# Autodesk Inventor assembly: Planktoscope_Mini_v0
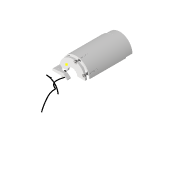
[picture p0: Inventor's stored thumbnail of the model, 180x180]
Saved by Autodesk Inventor 2022 (Build 260153000, 153)
## iProperties
Created: 2022-04-02
Part Number: Planktoscope_Mini_v0
Document SubType Name: Assembly
Designer: Prakash Lab
Author: Prakash Lab
## Documents named in this file (13)
- C:\Users\diederichbenedict\Dropbox\Dokumente\Promotion\PROJECTS\Matchboxscope\INVENTOR\Planktoscope_Mini\Planktoscope_Mini_v0.iam
- C:\Users\diederichbenedict\Dropbox\Dokumente\Promotion\PROJECTS\Matchboxscope\INVENTOR\MATCHBOXSCOPE\Matchboxscope_bottom_v0.ipt
- C:\Users\diederichbenedict\Dropbox\Dokumente\Promotion\PROJECTS\Matchboxscope\INVENTOR\MATCHBOXSCOPE\00_ESP3-CAM.iam
- C:\Users\diederichbenedict\Dropbox\Dokumente\Promotion\PROJECTS\Matchboxscope\INVENTOR\MATCHBOXSCOPE\00_Powerbank.ipt
- C:\Users\diederichbenedict\Dropbox\Dokumente\Promotion\PROJECTS\Matchboxscope\INVENTOR\MATCHBOXSCOPE\00_spring.ipt
- C:\Users\diederichbenedict\Documents\Inventor\Content Center Files\R2022\de-DE\DIN 912\DIN 912 - M3 x 0.5 x 25 x 18.ipt
- C:\Users\diederichbenedict\Dropbox\Dokumente\Promotion\PROJECTS\Matchboxscope\INVENTOR\MATCHBOXSCOPE\Matchboxscope_middle2_v2.ipt
- C:\Users\diederichbenedict\Dropbox\Dokumente\Promotion\PROJECTS\Matchboxscope\INVENTOR\MATCHBOXSCOPE\Anglerfish_Cameraspacer.ipt
- C:\Users\diederichbenedict\Dropbox\Dokumente\Promotion\PROJECTS\Matchboxscope\INVENTOR\MATCHBOXSCOPE\Matchboxscope_sample_universal_toslink.ipt
- C:\Users\diederichbenedict\Dropbox\Dokumente\Promotion\PROJECTS\Matchboxscope\INVENTOR\MATCHBOXSCOPE\Planktoscope_Mini_Peristalticpump.iam
- C:\Users\diederichbenedict\Dropbox\Dokumente\Promotion\PROJECTS\Matchboxscope\INVENTOR\Planktoscope_Mini\00_Toslink.ipt
- C:\Users\diederichbenedict\Dropbox\Dokumente\Promotion\PROJECTS\Matchboxscope\INVENTOR\MATCHBOXSCOPE\Planktoscope_Mini_Electronicbase.iam
- C:\Users\diederichbenedict\Dropbox\Dokumente\Promotion\PROJECTS\Matchboxscope\INVENTOR\MATCHBOXSCOPE\Planktoscope_connectortube.ipt
## Components (20 placed, 12 different names)
1. Matchboxscope_bottom_v0:1 — Mate:1, Mate:2, Mate:3, Mate:4, Flush:1, Einfügen:1, Winkel:1, Passend:8, Passend:9
2. 00_ESP3-CAM:1 [sub-assembly] — Mate:4, Flush:1, Passend:5
3. 00_Powerbank:1
4. 00_spring:1
5. DIN 912 - ersetzt durch DIN EN ISO 4762 M3 x 25:1 — Passend:6
6. DIN 912 - ersetzt durch DIN EN ISO 4762 M3 x 25:2
7. DIN 912 - ersetzt durch DIN EN ISO 4762 M3 x 25:3
8. 00_spring:3
9. 00_spring:4
10. DIN 912 - ersetzt durch DIN EN ISO 4762 M3 x 25:4
11. DIN 912 - ersetzt durch DIN EN ISO 4762 M3 x 25:5
12. DIN 912 - ersetzt durch DIN EN ISO 4762 M3 x 25:6
13. DIN 912 - ersetzt durch DIN EN ISO 4762 M3 x 25:7
14. Matchboxscope_middle2_v2:1 — Einfügen:1, Passend:5, Winkel:1, Passend:7
15. Anglerfish_Cameraspacer:1
16. Matchboxscope_sample_universal_toslink:1 — Passend:6, Passend:7, Einfügen:2
17. Planktoscope_Mini_Peristalticpump:1 [sub-assembly] — Passend:8, Passend:9, Fluchtend:6, Fluchtend:7
18. 00_Toslink:1 — Einfügen:2
19. Planktoscope_Mini_Electronicbase:2 [sub-assembly]
20. Planktoscope_connectortube:1 — Fluchtend:6, Fluchtend:7
## Relationships (22: Mate 12, Flush 7, Insert 2, Angle 1)
- Mate:1: Matchboxscope_bottom_v0:1
- Mate:2: Matchboxscope_bottom_v0:1
- Mate:3: Matchboxscope_bottom_v0:1
- Mate:4: Matchboxscope_bottom_v0:1 ↔ 00_ESP3-CAM:1
- Flush:1: Matchboxscope_bottom_v0:1 ↔ 00_ESP3-CAM:1
- Einfügen:1 [Insert]: Matchboxscope_bottom_v0:1 ↔ Matchboxscope_middle2_v2:1
- Passend:5 [Mate] (3 mm): 00_ESP3-CAM:1 ↔ Matchboxscope_middle2_v2:1
- Winkel:1 [Angle] (180 deg): Matchboxscope_bottom_v0:1 ↔ Matchboxscope_middle2_v2:1
- Passend:6 [Mate]: DIN 912 - ersetzt durch DIN EN ISO 4762 M3 x 25:1 ↔ Matchboxscope_sample_universal_toslink:1
- Passend:7 [Mate]: Matchboxscope_middle2_v2:1 ↔ Matchboxscope_sample_universal_toslink:1
- Passend:8 [Mate]: Matchboxscope_bottom_v0:1 ↔ Planktoscope_Mini_Peristalticpump:1
- Passend:9 [Mate]: Matchboxscope_bottom_v0:1 ↔ Planktoscope_Mini_Peristalticpump:1
- Einfügen:2 [Insert] (12 mm): Matchboxscope_sample_universal_toslink:1 ↔ 00_Toslink:1
- [Mate] (3 mm): Planktoscope_Mini_Peristalticpump:1 ↔ Planktoscope_Mini_Electronicbase:2
- [Mate]: Planktoscope_Mini_Peristalticpump:1 ↔ Planktoscope_Mini_Electronicbase:2
- [Mate]: Planktoscope_Mini_Peristalticpump:1 ↔ Planktoscope_Mini_Electronicbase:2
- [Flush]: Planktoscope_Mini_Peristalticpump:1 ↔ Planktoscope_Mini_Electronicbase:2
- [Flush]: Planktoscope_Mini_Peristalticpump:1 ↔ Planktoscope_Mini_Electronicbase:2
- [Flush]: Planktoscope_Mini_Peristalticpump:1 ↔ Planktoscope_Mini_Electronicbase:2
- [Flush]: Planktoscope_Mini_Peristalticpump:1 ↔ Planktoscope_Mini_Electronicbase:2
- Fluchtend:6 [Flush]: Planktoscope_Mini_Peristalticpump:1 ↔ Planktoscope_connectortube:1
- Fluchtend:7 [Flush]: Planktoscope_Mini_Peristalticpump:1 ↔ Planktoscope_connectortube:1
